# Autodesk Inventor assembly: aerogelInHolder
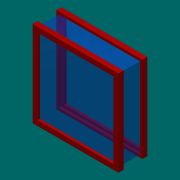
[picture p0: Inventor's stored thumbnail of the model, 180x180]
Saved by Autodesk Inventor 2016 (Build 200138000, 138)
## iProperties
Created: 2015-10-27
Part Number: aerogelInHolder
Document SubType Name: Assembly
Designer: Sawaiz
Author: Sawaiz
## Documents named in this file (3)
- C:\Users\Sawaiz\OneDrive\projects\modularRICH\aerogel\aerogelInHolder.iam
- C:\Users\Sawaiz\OneDrive\projects\modularRICH\aerogel\aerogelBlock.ipt
- C:\Users\Sawaiz\OneDrive\projects\modularRICH\aerogel\aerogelHolder.ipt
## Components (3 placed, 2 different names)
1. aerogelBlock:1 — Mate:1, Mate:2, Mate:3, Mate:4
2. aerogelHolder:1 — Flush:1, Flush:2, Mate:1, Mate:3
3. aerogelHolder:2 — Flush:1, Flush:2, Mate:2, Mate:4
## Relationships (6: Mate 4, Flush 2)
- Flush:1: aerogelHolder:1 ↔ aerogelHolder:2
- Flush:2: aerogelHolder:1 ↔ aerogelHolder:2
- Mate:1: aerogelBlock:1 ↔ aerogelHolder:1
- Mate:2: aerogelBlock:1 ↔ aerogelHolder:2
- Mate:3: aerogelBlock:1 ↔ aerogelHolder:1
- Mate:4: aerogelBlock:1 ↔ aerogelHolder:2
